# Autodesk Inventor assembly: SUMEC_Box
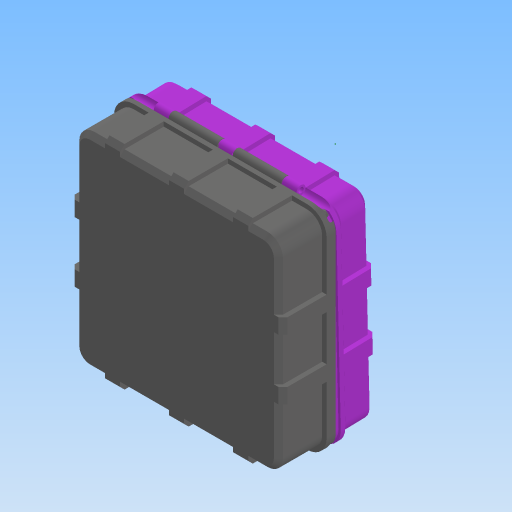
[picture p0: Inventor's stored thumbnail of the model, 512x512]
Saved by Autodesk Inventor 2024 (Build 280153000, 153)
## iProperties
Created: 2024-03-01
Part Number: SUMEC_Box
Document SubType Name: Assembly
Designer: MenMe
Author: MenMe
## Documents named in this file (3)
- C:\Users\MenMe\Documents\GitHub\RoboCop\- 3D -\_wip\SUMEC_Box.iam
- C:\Users\MenMe\Documents\GitHub\RoboCop\- 3D -\_wip\SUMEC_box.ipt
- C:\Users\MenMe\Documents\GitHub\RoboCop\- 3D -\_wip\SUMEC_box_top.ipt
## Components (2 placed, 2 different names)
1. SUMEC_box:1 — Rotational:1
2. SUMEC_box_top:1 — Rotational:1
## Relationships (1: RevoluteJoint 1)
- Rotational:1 [RevoluteJoint]: SUMEC_box:1 ↔ SUMEC_box_top:1
